# Autodesk Inventor assembly: 2016-01-23-RhinoRobot
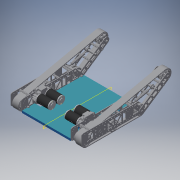
[picture p0: Inventor's stored thumbnail of the model, 180x180]
Saved by Autodesk Inventor 2016 SP1 (Build 200210100, 210)
## iProperties
Created: 2016-01-23
Part Number: 2016-01-23-RhinoRobot
Document SubType Name: Assembly
Designer: steele
Author: steele
## Documents named in this file (5)
- C:\snobotics\CAD-Development\robSteele\SnoBotics2016\2016-01-23-RhinoRobot\2016-01-23-RhinoRobot.iam
- C:\snobotics\CAD-Development\robSteele\SnoBotics2016\RhinoBottomFloorOptions\RhinoBottomFloorPlate01.ipt
- C:\snobotics\CAD-Development\robSteele\SnoBotics2016\RhinoTrackDriveModule\am-3322+RhinoTrackDriveModule.iam
- C:\snobotics\CAD-Development\robSteele\SnoBotics2016\RhinoBottomFloorOptions\RhinoBottomFloorPlate01_MIR1.ipt
- C:\snobotics\CAD-Development\robSteele\SnoBotics2016\RhinoTrackDriveModule\am-3322+RhinoTrackDriveModule_MIR.iam
## Components (4 placed, 4 different names)
1. RhinoBottomFloorPlate01:1 — Mate:1, Flush:1, Flush:2
2. am-3322+RhinoTrackDriveModule:1 [sub-assembly] — Mate:1, Flush:1, Flush:2
3. RhinoBottomFloorPlate01_MIR1:1 — Mate:2, Flush:3, Flush:4
4. am-3322+RhinoTrackDriveModule_MIR:1 [sub-assembly] — Mate:2, Flush:3, Flush:4
## Relationships (6: Flush 4, Mate 2)
- Mate:1 (3.175 mm): RhinoBottomFloorPlate01:1 ↔ am-3322+RhinoTrackDriveModule:1
- Flush:1: RhinoBottomFloorPlate01:1 ↔ am-3322+RhinoTrackDriveModule:1
- Flush:2: RhinoBottomFloorPlate01:1 ↔ am-3322+RhinoTrackDriveModule:1
- Mate:2 (3.175 mm): RhinoBottomFloorPlate01_MIR1:1 ↔ am-3322+RhinoTrackDriveModule_MIR:1
- Flush:3: RhinoBottomFloorPlate01_MIR1:1 ↔ am-3322+RhinoTrackDriveModule_MIR:1
- Flush:4: RhinoBottomFloorPlate01_MIR1:1 ↔ am-3322+RhinoTrackDriveModule_MIR:1
## Named parameters: robotWidth = 609.6 mm, halfRobotWidth = 304.8 mm, maxPerimeter = 3048 mm, maxLength = 914.4 mm, widthOfTrack = 95.25 mm, boardWidth = 419.1 mm
